# Autodesk Inventor assembly: Assembly
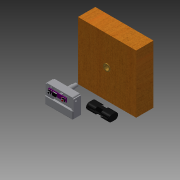
[picture p0: Inventor's stored thumbnail of the model, 180x180]
Saved by Autodesk Inventor 2014 (Build 180170000, 170)
## iProperties
Created: 2014-05-02
Part Number: Assembly
Document SubType Name: Assembly
Designer: Alex
Author: Alex
## Documents named in this file (7)
- C:\Users\Alex\Desktop\LEDStatusIndicator\Assembly.iam
- C:\Users\Alex\Desktop\LEDStatusIndicator\Case_Cutout.ipt
- C:\Users\Alex\Desktop\LEDStatusIndicator\Tube_Part.ipt
- C:\Users\Alex\Desktop\LEDStatusIndicator\Back_Shield.ipt
- C:\Users\Alex\Desktop\LEDStatusIndicator\Battery Pack.ipt
- C:\Users\Alex\Desktop\LEDStatusIndicator\Door.ipt
- C:\Users\Alex\Desktop\LEDStatusIndicator\LED Indicator.ipt
## Components (6 placed, 6 different names)
1. Case_Cutout:1 — Mate:1, Mate:2, Mate:3, Mate:4, Mate:5, Mate:6, Flush:2, Flush:3
2. Tube_Part:1 — Mate:1, Mate:2, Mate:3, Mate:7, Mate:8
3. Back_Shield:1 — Mate:4, Mate:5, Mate:6, Flush:1, Flush:4
4. Battery Pack:1
5. Door:1 — Mate:7, Flush:1, Flush:2
6. LED Indicator:1 — Mate:8, Flush:3, Flush:4
## Relationships (12: Mate 8, Flush 4)
- Mate:1: Case_Cutout:1 ↔ Tube_Part:1
- Mate:2: Case_Cutout:1 ↔ Tube_Part:1
- Mate:3: Case_Cutout:1 ↔ Tube_Part:1
- Mate:4: Case_Cutout:1 ↔ Back_Shield:1
- Mate:5: Case_Cutout:1 ↔ Back_Shield:1
- Mate:6: Case_Cutout:1 ↔ Back_Shield:1
- Mate:7: Tube_Part:1 ↔ Door:1
- Flush:1 (39.37 mm): Back_Shield:1 ↔ Door:1
- Flush:2 (66.04 mm): Case_Cutout:1 ↔ Door:1
- Mate:8: Tube_Part:1 ↔ LED Indicator:1
- Flush:3 (5.08 mm): Case_Cutout:1 ↔ LED Indicator:1
- Flush:4 (15.24 mm): Back_Shield:1 ↔ LED Indicator:1
